# Autodesk Inventor assembly: LegEncoderBoard
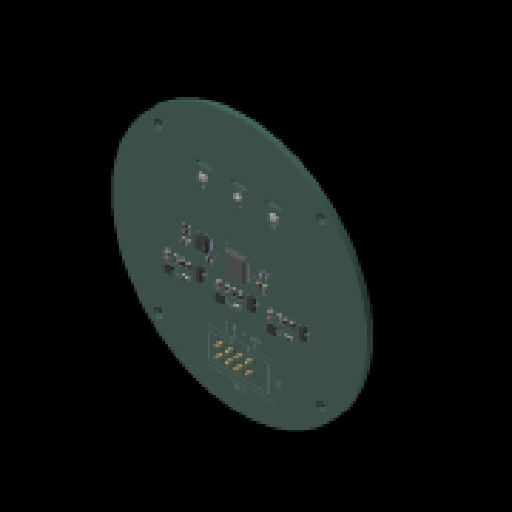
[picture p0: Inventor's stored thumbnail of the model, 512x512]
Saved by Autodesk Inventor 2025.2 (Build 292293000, 293)
## iProperties
Company: Kicad
Created: 2026-02-13
Part Number: LegEncoderBoard
Description: KiCad electronic assembly
Document SubType Name: Assembly
Designer: valer
Authority: Unknown
Sending System: KiCad to STEP converter
Preprocessor: Open CASCADE STEP processor 7.8
Title: LegEncoderBoardLatest.step
Author: Pcbnew
## Documents named in this file (20)
- C:\Users\valer\Desktop\str1ker\cad\external\WheelEncoder\WheelEncoderBoard.iam
- C:\Users\valer\Desktop\str1ker\cad\external\WheelEncoder\CC0603JRX7R7BB105.ipt
- C:\Users\valer\Desktop\str1ker\cad\external\WheelEncoder\RC0603FR-0722RL.ipt
- C:\Users\valer\Desktop\str1ker\cad\external\WheelEncoder\RCG06031K00FKEA.ipt
- C:\Users\valer\Desktop\str1ker\cad\external\WheelEncoder\RC0603FR-07150RL.ipt
- C:\Users\valer\Desktop\str1ker\cad\external\WheelEncoder\RC0603FR-07470KL.ipt
- C:\Users\valer\Desktop\str1ker\cad\external\WheelEncoder\BAT54WS-7-F.ipt
- C:\Users\valer\Desktop\str1ker\cad\external\WheelEncoder\GRM1885C1H103JA01D.ipt
- C:\Users\valer\Desktop\str1ker\cad\external\WheelEncoder\TSSOP-14_AMS.ipt
- C:\Users\valer\Desktop\str1ker\cad\external\WheelEncoder\CC0603KRX7R9BB104.ipt
- C:\Users\valer\Desktop\str1ker\cad\external\WheelEncoder\IDC-Header_2x04_P2.54mm_Vertical.ipt
- C:\Users\valer\Desktop\str1ker\cad\external\WheelEncoder\SN74LVC3G17DCTR.ipt
- C:\Users\valer\Desktop\str1ker\cad\external\WheelEncoder\MMBT3904LT1G.ipt
- C:\Users\valer\Desktop\str1ker\cad\external\WheelEncoder\150080BS75000.iam
- C:\Users\valer\Desktop\str1ker\cad\external\WheelEncoder\NCD0603R1.iam
- C:\Users\valer\Desktop\str1ker\cad\external\WheelEncoder\CRCW0603100KFKEA.ipt
- C:\Users\valer\Desktop\str1ker\cad\external\WheelEncoder\RC0603FR-0747KL.ipt
- C:\Users\valer\Desktop\str1ker\cad\external\WheelEncoder\LegEncoderBoard_silkscreen.ipt
- C:\Users\valer\Desktop\str1ker\cad\external\WheelEncoder\LegEncoderBoard_silkscreen_1.ipt
- C:\Users\valer\Desktop\str1ker\cad\external\WheelEncoder\LegEncoderBoard_PCB.ipt
## Components (37 placed, 37 different names)
1. 1
2. 2
3. 3
4. 4
5. 5
6. 6
7. 7
8. 8
9. 9
10. 10
11. 11
12. 12
13. 13
14. IdcConnector — Mate:1, Flush:1
15. 15
16. 16
17. 23 [sub-assembly]
18. 29 [sub-assembly]
19. 30
20. 31
21. 32
22. 33
23. 34
24. 35
25. 36
26. 37 [sub-assembly]
27. 38
28. 39
29. 40
30. 41
31. 42
32. 43
33. 44
34. 45
35. 46
36. 47
37. Board — Mate:1, Flush:1
## Relationships (2: Mate 1, Flush 1)
- Mate:1: IdcConnector ↔ Board
- Flush:1: IdcConnector ↔ Board
